# Autodesk Inventor assembly: CARRO
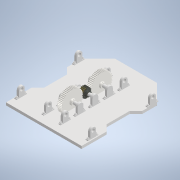
[picture p0: Inventor's stored thumbnail of the model, 180x180]
Saved by Autodesk Inventor 2021 (Build 250183000, 183)
## iProperties
Created: 2021-02-07
Part Number: CARRO
Document SubType Name: Assembly
Designer: rotje
Author: rotje
## Documents named in this file (4)
- C:\Users\rotje\Documents\Inventor\MSF\CARRO.iam
- C:\Users\rotje\Documents\Inventor\MSF\Base-soporte.iam
- C:\Users\rotje\Documents\Inventor\MSF\Eje-engrane.iam
- C:\Users\rotje\Documents\Inventor\MSF\Eje-engrane_chico.iam
## Components (4 placed, 3 different names)
1. Base-soporte:1 [sub-assembly] — Insertar:1, Insertar:2, Insertar:3, Coincidencia:1
2. Eje-engrane:1 [sub-assembly] — Insertar:3
3. Eje-engrane:2 [sub-assembly] — Insertar:1
4. Eje-engrane_chico:1 [sub-assembly] — Insertar:2
## Relationships (4: Insert 3, Mate 1)
- Insertar:1: Base-soporte:1 ↔ Eje-engrane:2
- Insertar:2: Base-soporte:1 ↔ Eje-engrane_chico:1
- Insertar:3: Base-soporte:1 ↔ Eje-engrane:1
- Coincidencia:1 [Mate]: Base-soporte:1
